# Autodesk Inventor assembly: kuckle-join-Assembly
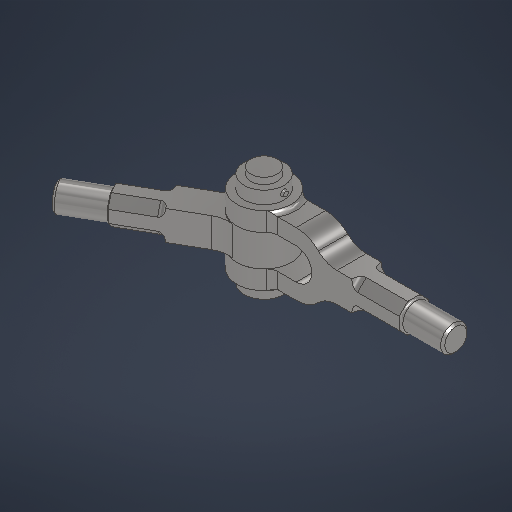
[picture p0: Inventor's stored thumbnail of the model, 512x512]
Saved by Autodesk Inventor 2026.1 (Build 301233020, 233B)
## iProperties
Created: 2025-12-18
Part Number: kuckle-join-Assembly
Document SubType Name: Assembly
Designer: kngob
Author: kngob
## Documents named in this file (6)
- C:\Users\kngob\projects\Inventor\knuckle-joint\kuckle-join-Assembly.iam
- C:\Users\kngob\projects\Inventor\knuckle-joint\fork-end.ipt
- C:\Users\kngob\projects\Inventor\knuckle-joint\eye-end.ipt
- C:\Users\kngob\projects\Inventor\knuckle-joint\pin.ipt
- C:\Users\kngob\projects\Inventor\knuckle-joint\collar.ipt
- C:\Users\kngob\projects\Inventor\knuckle-joint\pin-2.ipt
## Components (5 placed, 5 different names)
1. fork-end:1 — Flush:1, Mate:1, Mate:2, Mate:3, Mate:4, Mate:5, Mate:6, Mate:8
2. eye-end:1 — Mate:3, Mate:4
3. pin:1 — Mate:5, Mate:6, Mate:7, Mate:9
4. collar:1 — Mate:7, Mate:8, Mate:9, Mate:10, Tangent:1
5. pin-2:1 — Mate:10, Tangent:1
## Relationships (12: Mate 10, Flush 1, Tangent 1)
- Flush:1: fork-end:1
- Mate:1: fork-end:1
- Mate:2: fork-end:1
- Mate:3: fork-end:1 ↔ eye-end:1
- Mate:4: fork-end:1 ↔ eye-end:1
- Mate:5: fork-end:1 ↔ pin:1
- Mate:6: fork-end:1 ↔ pin:1
- Mate:7: pin:1 ↔ collar:1
- Mate:8: fork-end:1 ↔ collar:1
- Mate:9: pin:1 ↔ collar:1
- Mate:10: collar:1 ↔ pin-2:1
- Tangent:1: collar:1 ↔ pin-2:1
